# Autodesk Inventor assembly: WE5x2
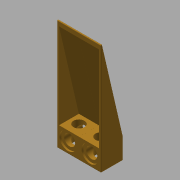
[picture p0: Inventor's stored thumbnail of the model, 180x180]
Saved by Autodesk Inventor 2019.3 (Build 233278000, 278)
## iProperties
Created: 2019-02-07
Part Number: WE5x2
Document SubType Name: Assembly
Designer: Varga Daniel
Author: Varga Daniel
Wedge_assembly_length: 50,000 mm
## Documents named in this file (5)
- C:\!_Dani\!_cloud\OneDrive\!_munka\Revolution\RevvyDemoKit\Structural parts\Wedges\WE2+x1+\WE5x2.iam
- C:\!_Dani\!_cloud\OneDrive\!_munka\Revolution\RevvyDemoKit\Structural parts\Wedges\Wedge_base.ipt
- C:\!_Dani\!_cloud\OneDrive\!_munka\Revolution\RevvyDemoKit\Structural parts\Wedges\Wedge_base\Wedge_base-right.ipt
- C:\!_Dani\!_cloud\OneDrive\!_munka\Revolution\RevvyDemoKit\Structural parts\Wedges\Wedge_base\Wedge_base-left.ipt
- C:\!_Dani\!_cloud\OneDrive\!_munka\Revolution\RevvyDemoKit\Structural parts\Wedges\WE2+x1+.iam
## Components (2 placed, 2 different names)
1. Wedge_base-left:1 — Flush:2, Flush:4, Mate:1
2. Wedge_base-right:2 — Flush:2, Flush:4, Mate:1
## Relationships (3: Flush 2, Mate 1)
- Flush:2: Wedge_base-left:1 ↔ Wedge_base-right:2
- Flush:4: Wedge_base-left:1 ↔ Wedge_base-right:2
- Mate:1: Wedge_base-left:1 ↔ Wedge_base-right:2
